# Autodesk Inventor assembly: VersaBlock Assembly
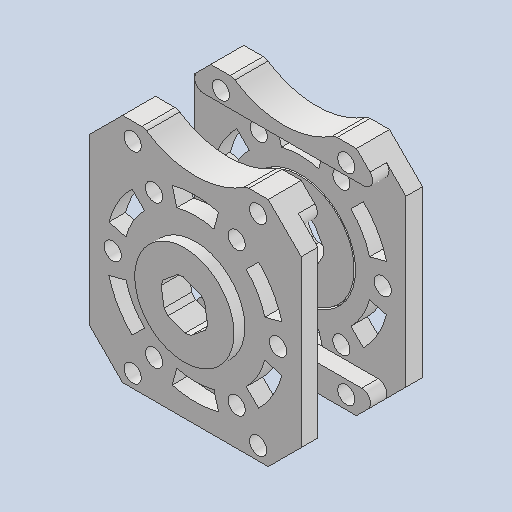
[picture p0: Inventor's stored thumbnail of the model, 512x512]
Saved by Autodesk Inventor 2022 (Build 260153000, 153)
## iProperties
Created: 2020-01-16
Part Number: VersaBlock Assembly
Document SubType Name: Assembly
Designer: aidan
Author: aidan
## Documents named in this file (3)
- C:\Users\Ty Gazaway\Documents\t3-cad\CAD\VersaBlock Assembly.iam
- C:\Users\Ty Gazaway\Documents\t3-cad\CAD\Versa Chassis Bearing Block.ipt
- C:\Users\Ty Gazaway\Documents\t3-cad\CAD\Bearing for THUNDER.ipt
## Components (4 placed, 2 different names)
1. Versa Chassis Bearing Block:1 — Flush:1, Flush:2, Mate:1, Insert:2
2. Versa Chassis Bearing Block:2 — Flush:1, Flush:2, Mate:1, Insert:1
3. Bearing for THUNDER:1 — Insert:2
4. Bearing for THUNDER:2 — Insert:1
## Relationships (5: Flush 2, Insert 2, Mate 1)
- Flush:1: Versa Chassis Bearing Block:1 ↔ Versa Chassis Bearing Block:2
- Flush:2: Versa Chassis Bearing Block:1 ↔ Versa Chassis Bearing Block:2
- Mate:1 (25.4 mm): Versa Chassis Bearing Block:1 ↔ Versa Chassis Bearing Block:2
- Insert:1: Versa Chassis Bearing Block:2 ↔ Bearing for THUNDER:2
- Insert:2: Versa Chassis Bearing Block:1 ↔ Bearing for THUNDER:1
